# Autodesk Inventor assembly: 3d_LM-Welding_Tooling - Lathe carriage
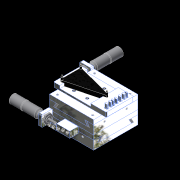
[picture p0: Inventor's stored thumbnail of the model, 180x180]
Saved by Autodesk Inventor 2018.3 (Build 223284000, 284)
## iProperties
Created: 2026-02-27
Part Number: 3d_LM-Welding_Tooling - Lathe carriage
Document SubType Name: Assembly
Designer: aca6
Author: aca6
## Documents named in this file (19)
- C:\Users\aca6\git\LM\items\3d_LM\items\LM-Welding_Tooling\3d_LM-Welding_Tooling\3d\3d_LM-Welding_Tooling - Lathe carriage.iam
- C:\Users\aca6\git\LM\items\3d_LM\items\LM-Welding_Tooling\3d_LM-Welding_Tooling\3d\3d_LM-Welding_Tooling - Adapter.ipt
- C:\Users\aca6\git\LM\items\3d_LM\items\LM-Welding_Tooling\3d_LM-Welding_Tooling\3d\3d_LM-Welding_Tooling -  Guide Pin.ipt
- C:\Users\aca6\git\LM\items\3d_LM\items\LM-Welding_Tooling\3d_LM-Welding_Tooling\3d\3d_LM-Welding_Tooling - Top Adapter.ipt
- C:\Users\aca6\git\LM\items\3d_LM\items\LM-Welding_Tooling\3d_LM-Welding_Tooling\3d\3d_LM-Welding_Tooling -  Moving Block.ipt
- C:\Users\aca6\git\LM\items\3d_LM\items\LM-Welding_Tooling\3d_LM-Welding_Tooling\3d\3d_LM-Welding_Tooling - Fixed base.ipt
- C:\Users\aca6\git\LM\items\3d_LM\items\LM-Welding_Tooling\3d_LM-Welding_Tooling\3d\3d_LM-Welding_Tooling - Acetal Stick.ipt
- C:\Users\aca6\git\LM\items\3d_LM\items\LM-Welding_Tooling\3d_LM-Welding_Tooling\3d\3d_LM-Welding_Tooling - Upper fixed base.ipt
- C:\Users\aca6\git\LM\items\3d_LM\items\LM-Welding_Tooling\3d_LM-Welding_Tooling\3d\3d_LM-Welding_Tooling - Upper moving base.ipt
- C:\Users\aca6\git\LM\items\_accesories\Tornilleria\Tornillos\3d_DIN 7991\3d\A4 Black Inox\DIN 7991 - M3x14 Black INOX.ipt
- C:\Users\aca6\git\LM\items\_accesories\Tornilleria\Tornillos\3d_DIN 7991\3d\A4 Black Inox\DIN 7991 - M3x12 Black INOX.ipt
- C:\Users\aca6\git\LM\items\3d_LM\items\LM-Welding_Tooling\3d_LM-Welding_Tooling\3d\3d_LM-Welding_Tooling -  Micrometer Nut.ipt
- C:\Users\aca6\git\LM\items\3d_LM\items\LM-Welding_Tooling\3d_LM-Welding_Tooling\3d\3d_LM-Welding_Tooling -  Micrometer.ipt
- C:\Users\aca6\git\LM\items\3d_LM\items\LM-Welding_Tooling\3d_LM-Welding_Tooling\3d\3d_LM-Welding_Tooling - Fixed Block.ipt
- C:\Users\aca6\git\LM\items\_accesories\Tornilleria\Tornillos\3d_Accu Group\3d\Prisionero nylon M4x7 REF SSN-M4-7.ipt
- C:\Users\aca6\git\LM\items\_accesories\Tornilleria\Tornillos\3d_DIN 912\3d\A4 Inox\DIN 912 - M3 x 0,5 x 8 -  INOX.ipt
- C:\Users\aca6\git\LM\items\_accesories\Tornilleria\Tornillos\3d_DIN 912\3d\A4 Inox\DIN 912 - M3 x 0,5 x 30 -  INOX.ipt
- C:\Users\aca6\git\LM\items\_accesories\Tornilleria\Tornillos\3d_DIN 912\3d\A4 Inox\DIN 912 - M3 x 0,5 x 10 -  INOX.ipt
- C:\Users\aca6\git\LM\items\3d_LM\items\LM-Welding_Tooling\3d_LM-Welding_Tooling\3d\3d_LM-Welding_Tooling - Moving base.ipt
## Components (51 placed, 18 different names)
1. 3d_LM-Welding_Tooling - Adapter:1
2. 3d_LM-Welding_Tooling -  Guide Pin:1
3. 3d_LM-Welding_Tooling -  Guide Pin:2
4. 3d_LM-Welding_Tooling -  Guide Pin:3
5. 3d_LM-Welding_Tooling - Top Adapter:1
6. 3d_LM-Welding_Tooling - Fixed base:1 — Mate:83, Flush:28, Mate:84, Flush:29
7. 3d_LM-Welding_Tooling - Acetal Stick:1 — Mate:83, Flush:28, Mate:85
8. 3d_LM-Welding_Tooling - Acetal Stick:2
9. 3d_LM-Welding_Tooling - Upper fixed base:1 — Mate:80, Mate:81, Mate:82
10. 3d_LM-Welding_Tooling - Acetal Stick:3
11. 3d_LM-Welding_Tooling - Acetal Stick:4
12. 3d_LM-Welding_Tooling - Upper moving base:1 — Flush:29
13. DIN 7991 - M3x14 Black INOX:1
14. DIN 7991 - M3x14 Black INOX:2
15. DIN 7991 - M3x14 Black INOX:3
16. DIN 7991 - M3x14 Black INOX:4
17. DIN 7991 - M3x12 Black INOX:1
18. DIN 7991 - M3x12 Black INOX:2
19. DIN 7991 - M3x12 Black INOX:3
20. DIN 7991 - M3x12 Black INOX:4
21. 3d_LM-Welding_Tooling -  Micrometer Nut:1
22. 3d_LM-Welding_Tooling -  Micrometer:1
23. 3d_LM-Welding_Tooling -  Micrometer Nut:2
24. 3d_LM-Welding_Tooling - Fixed Block:1
25. 3d_LM-Welding_Tooling -  Moving Block:3
26. Prisionero nylon M4x7 REF SSN-M4-7:1
27. Prisionero nylon M4x7 REF SSN-M4-7:2
28. Prisionero nylon M4x7 REF SSN-M4-7:3
29. Prisionero nylon M4x7 REF SSN-M4-7:4
30. 3d_LM-Welding_Tooling - Fixed Block:2
31. 3d_LM-Welding_Tooling -  Micrometer:2
32. 3d_LM-Welding_Tooling -  Moving Block:4
33. Prisionero nylon M4x7 REF SSN-M4-7:5
34. Prisionero nylon M4x7 REF SSN-M4-7:6
35. Prisionero nylon M4x7 REF SSN-M4-7:7
36. Prisionero nylon M4x7 REF SSN-M4-7:8
37. Prisionero nylon M4x7 REF SSN-M4-7:9
38. Prisionero nylon M4x7 REF SSN-M4-7:10
39. Prisionero nylon M4x7 REF SSN-M4-7:11
40. Prisionero nylon M4x7 REF SSN-M4-7:12
41. DIN 912 - M3 x 0,5 x 8 -  INOX:1
42. DIN 912 - M3 x 0,5 x 8 -  INOX:2
43. DIN 912 - M3 x 0,5 x 30 -  INOX:1 — Mate:86
44. DIN 912 - M3 x 0,5 x 30 -  INOX:2
45. DIN 912 - M3 x 0,5 x 30 -  INOX:3
46. DIN 912 - M3 x 0,5 x 30 -  INOX:4
47. DIN 912 - M3 x 0,5 x 10 -  INOX:1
48. DIN 912 - M3 x 0,5 x 10 -  INOX:2
49. DIN 912 - M3 x 0,5 x 10 -  INOX:3
50. DIN 912 - M3 x 0,5 x 10 -  INOX:4
51. 3d_LM-Welding_Tooling - Moving base:1 — Mate:80, Mate:81, Mate:82, Mate:84, Mate:85, Mate:86
## Relationships (114: Mate 79, Flush 27, Tangent 8)
- [Mate]: 3d_LM-Welding_Tooling - Adapter:1 ↔ 3d_LM-Welding_Tooling -  Guide Pin:1
- [Mate]: 3d_LM-Welding_Tooling - Adapter:1 ↔ 3d_LM-Welding_Tooling -  Guide Pin:2
- [Mate]: 3d_LM-Welding_Tooling - Adapter:1 ↔ 3d_LM-Welding_Tooling -  Guide Pin:3
- [Mate]: 3d_LM-Welding_Tooling - Adapter:1 ↔ 3d_LM-Welding_Tooling -  Guide Pin:2
- [Mate]: 3d_LM-Welding_Tooling - Adapter:1 ↔ 3d_LM-Welding_Tooling -  Guide Pin:1
- [Mate]: 3d_LM-Welding_Tooling - Adapter:1 ↔ 3d_LM-Welding_Tooling -  Guide Pin:2
- [Mate]: 3d_LM-Welding_Tooling - Adapter:1 ↔ 3d_LM-Welding_Tooling -  Guide Pin:1
- [Mate]: 3d_LM-Welding_Tooling - Adapter:1 ↔ 3d_LM-Welding_Tooling -  Guide Pin:3
- [Flush]: 3d_LM-Welding_Tooling - Adapter:1 ↔ 3d_LM-Welding_Tooling - Top Adapter:1
- [Mate]: 3d_LM-Welding_Tooling -  Guide Pin:2 ↔ 3d_LM-Welding_Tooling - Top Adapter:1
- [Mate]: 3d_LM-Welding_Tooling -  Guide Pin:1 ↔ 3d_LM-Welding_Tooling - Top Adapter:1
- [Mate]: 3d_LM-Welding_Tooling - Fixed base:1 ↔ 3d_LM-Welding_Tooling - Acetal Stick:2
- [Mate]: 3d_LM-Welding_Tooling - Fixed base:1 ↔ 3d_LM-Welding_Tooling - Acetal Stick:2
- [Flush]: 3d_LM-Welding_Tooling - Fixed base:1 ↔ 3d_LM-Welding_Tooling - Acetal Stick:1
- [Flush]: 3d_LM-Welding_Tooling - Fixed base:1 ↔ 3d_LM-Welding_Tooling - Acetal Stick:2
- [Mate]: 3d_LM-Welding_Tooling - Upper fixed base:1 ↔ 3d_LM-Welding_Tooling - Acetal Stick:3
- [Mate]: 3d_LM-Welding_Tooling - Upper fixed base:1 ↔ 3d_LM-Welding_Tooling - Acetal Stick:3
- [Mate]: 3d_LM-Welding_Tooling - Upper fixed base:1 ↔ 3d_LM-Welding_Tooling - Acetal Stick:4
- [Mate]: 3d_LM-Welding_Tooling - Upper fixed base:1 ↔ 3d_LM-Welding_Tooling - Acetal Stick:4
- [Flush]: 3d_LM-Welding_Tooling - Upper fixed base:1 ↔ 3d_LM-Welding_Tooling - Acetal Stick:4
- [Flush]: 3d_LM-Welding_Tooling - Upper fixed base:1 ↔ 3d_LM-Welding_Tooling - Acetal Stick:3
- [Mate]: 3d_LM-Welding_Tooling - Upper fixed base:1 ↔ 3d_LM-Welding_Tooling - Upper moving base:1
- [Mate]: 3d_LM-Welding_Tooling - Acetal Stick:4 ↔ 3d_LM-Welding_Tooling - Upper moving base:1
- [Mate]: 3d_LM-Welding_Tooling - Upper fixed base:1 ↔ DIN 7991 - M3x14 Black INOX:3
- [Mate]: 3d_LM-Welding_Tooling - Upper fixed base:1 ↔ DIN 7991 - M3x14 Black INOX:4
- [Mate]: 3d_LM-Welding_Tooling - Upper fixed base:1 ↔ DIN 7991 - M3x14 Black INOX:1
- [Mate]: 3d_LM-Welding_Tooling - Upper fixed base:1 ↔ DIN 7991 - M3x14 Black INOX:2
- [Tangent]: 3d_LM-Welding_Tooling - Upper fixed base:1 ↔ DIN 7991 - M3x14 Black INOX:4
- [Tangent]: 3d_LM-Welding_Tooling - Upper fixed base:1 ↔ DIN 7991 - M3x14 Black INOX:2
- [Tangent]: 3d_LM-Welding_Tooling - Upper fixed base:1 ↔ DIN 7991 - M3x14 Black INOX:1
- [Tangent]: 3d_LM-Welding_Tooling - Upper fixed base:1 ↔ DIN 7991 - M3x14 Black INOX:3
- [Mate]: 3d_LM-Welding_Tooling - Adapter:1 ↔ 3d_LM-Welding_Tooling - Upper moving base:1
- [Flush] (18.75 mm): 3d_LM-Welding_Tooling - Adapter:1 ↔ 3d_LM-Welding_Tooling - Upper moving base:1
- [Flush] (-9.684 mm): 3d_LM-Welding_Tooling - Adapter:1 ↔ 3d_LM-Welding_Tooling - Upper moving base:1
- [Mate]: 3d_LM-Welding_Tooling - Adapter:1 ↔ DIN 7991 - M3x12 Black INOX:4
- [Mate]: 3d_LM-Welding_Tooling - Adapter:1 ↔ DIN 7991 - M3x12 Black INOX:1
- [Mate]: 3d_LM-Welding_Tooling - Adapter:1 ↔ DIN 7991 - M3x12 Black INOX:3
- [Mate]: 3d_LM-Welding_Tooling - Adapter:1 ↔ DIN 7991 - M3x12 Black INOX:2
- [Tangent]: 3d_LM-Welding_Tooling - Adapter:1 ↔ DIN 7991 - M3x12 Black INOX:3
- [Tangent]: 3d_LM-Welding_Tooling - Adapter:1 ↔ DIN 7991 - M3x12 Black INOX:2
- [Tangent]: 3d_LM-Welding_Tooling - Adapter:1 ↔ DIN 7991 - M3x12 Black INOX:4
- [Tangent]: 3d_LM-Welding_Tooling - Adapter:1 ↔ DIN 7991 - M3x12 Black INOX:1
- [Mate]: 3d_LM-Welding_Tooling -  Micrometer:1 ↔ 3d_LM-Welding_Tooling - Fixed Block:1
- [Mate]: 3d_LM-Welding_Tooling -  Micrometer:1 ↔ 3d_LM-Welding_Tooling - Fixed Block:1
- [Mate]: 3d_LM-Welding_Tooling -  Micrometer:1 ↔ 3d_LM-Welding_Tooling -  Micrometer Nut:2
- [Mate]: 3d_LM-Welding_Tooling -  Micrometer Nut:2 ↔ 3d_LM-Welding_Tooling - Fixed Block:1
- [Mate]: 3d_LM-Welding_Tooling - Upper fixed base:1 ↔ 3d_LM-Welding_Tooling - Fixed Block:1
- [Flush]: 3d_LM-Welding_Tooling - Upper fixed base:1 ↔ 3d_LM-Welding_Tooling - Fixed Block:1
- [Mate]: 3d_LM-Welding_Tooling - Upper moving base:1 ↔ 3d_LM-Welding_Tooling -  Moving Block:3
- [Flush]: 3d_LM-Welding_Tooling - Upper fixed base:1 ↔ 3d_LM-Welding_Tooling - Upper moving base:1
- [Mate]: 3d_LM-Welding_Tooling - Upper fixed base:1 ↔ Prisionero nylon M4x7 REF SSN-M4-7:1
- [Mate]: 3d_LM-Welding_Tooling - Fixed base:1 ↔ Prisionero nylon M4x7 REF SSN-M4-7:2
- [Mate]: 3d_LM-Welding_Tooling - Upper fixed base:1 ↔ Prisionero nylon M4x7 REF SSN-M4-7:4
- [Mate]: 3d_LM-Welding_Tooling - Fixed base:1 ↔ Prisionero nylon M4x7 REF SSN-M4-7:3
- [Flush]: 3d_LM-Welding_Tooling - Fixed base:1 ↔ Prisionero nylon M4x7 REF SSN-M4-7:3
- [Flush]: 3d_LM-Welding_Tooling - Fixed base:1 ↔ Prisionero nylon M4x7 REF SSN-M4-7:2
- [Flush]: 3d_LM-Welding_Tooling - Upper fixed base:1 ↔ Prisionero nylon M4x7 REF SSN-M4-7:1
- [Flush]: 3d_LM-Welding_Tooling - Upper fixed base:1 ↔ Prisionero nylon M4x7 REF SSN-M4-7:4
- [Flush]: 3d_LM-Welding_Tooling - Upper fixed base:1 ↔ 3d_LM-Welding_Tooling - Fixed Block:1
- [Mate]: 3d_LM-Welding_Tooling - Fixed base:1 ↔ 3d_LM-Welding_Tooling - Fixed Block:2
- [Flush]: 3d_LM-Welding_Tooling - Fixed base:1 ↔ 3d_LM-Welding_Tooling - Fixed Block:2
- [Flush]: 3d_LM-Welding_Tooling - Fixed base:1 ↔ 3d_LM-Welding_Tooling - Fixed Block:2
- [Mate]: 3d_LM-Welding_Tooling - Fixed Block:2 ↔ 3d_LM-Welding_Tooling -  Micrometer:2
- [Mate]: 3d_LM-Welding_Tooling - Fixed Block:2 ↔ 3d_LM-Welding_Tooling -  Micrometer:2
- [Mate]: 3d_LM-Welding_Tooling -  Micrometer Nut:1 ↔ 3d_LM-Welding_Tooling -  Micrometer:2
- [Mate]: 3d_LM-Welding_Tooling -  Micrometer Nut:1 ↔ 3d_LM-Welding_Tooling - Fixed Block:2
- [Mate]: 3d_LM-Welding_Tooling - Upper moving base:1 ↔ Prisionero nylon M4x7 REF SSN-M4-7:5
- [Mate]: 3d_LM-Welding_Tooling - Upper moving base:1 ↔ Prisionero nylon M4x7 REF SSN-M4-7:8
- [Mate]: 3d_LM-Welding_Tooling - Upper moving base:1 ↔ Prisionero nylon M4x7 REF SSN-M4-7:7
- [Mate]: 3d_LM-Welding_Tooling - Upper moving base:1 ↔ Prisionero nylon M4x7 REF SSN-M4-7:6
- [Flush]: 3d_LM-Welding_Tooling - Upper moving base:1 ↔ Prisionero nylon M4x7 REF SSN-M4-7:6
- [Flush]: 3d_LM-Welding_Tooling - Upper moving base:1 ↔ Prisionero nylon M4x7 REF SSN-M4-7:5
- [Flush]: 3d_LM-Welding_Tooling - Upper moving base:1 ↔ Prisionero nylon M4x7 REF SSN-M4-7:7
- [Flush]: 3d_LM-Welding_Tooling - Upper moving base:1 ↔ Prisionero nylon M4x7 REF SSN-M4-7:8
- [Mate]: 3d_LM-Welding_Tooling - Fixed base:1 ↔ Prisionero nylon M4x7 REF SSN-M4-7:9
- [Flush]: 3d_LM-Welding_Tooling - Fixed base:1 ↔ Prisionero nylon M4x7 REF SSN-M4-7:9
- [Mate]: 3d_LM-Welding_Tooling - Fixed base:1 ↔ Prisionero nylon M4x7 REF SSN-M4-7:10
- [Flush]: 3d_LM-Welding_Tooling - Fixed base:1 ↔ Prisionero nylon M4x7 REF SSN-M4-7:10
- [Mate]: 3d_LM-Welding_Tooling - Upper fixed base:1 ↔ Prisionero nylon M4x7 REF SSN-M4-7:11
- [Flush]: 3d_LM-Welding_Tooling - Upper fixed base:1 ↔ Prisionero nylon M4x7 REF SSN-M4-7:11
- [Mate]: 3d_LM-Welding_Tooling - Upper fixed base:1 ↔ Prisionero nylon M4x7 REF SSN-M4-7:12
- [Flush]: 3d_LM-Welding_Tooling - Upper fixed base:1 ↔ Prisionero nylon M4x7 REF SSN-M4-7:12
- [Mate]: 3d_LM-Welding_Tooling -  Moving Block:4 ↔ DIN 912 - M3 x 0,5 x 8 -  INOX:2
- [Mate]: 3d_LM-Welding_Tooling -  Moving Block:4 ↔ DIN 912 - M3 x 0,5 x 8 -  INOX:2
- [Mate]: 3d_LM-Welding_Tooling -  Moving Block:3 ↔ DIN 912 - M3 x 0,5 x 8 -  INOX:1
- [Mate]: 3d_LM-Welding_Tooling -  Moving Block:3 ↔ DIN 912 - M3 x 0,5 x 8 -  INOX:1
- [Mate]: 3d_LM-Welding_Tooling -  Micrometer:2 ↔ 3d_LM-Welding_Tooling -  Moving Block:4
- [Mate]: 3d_LM-Welding_Tooling -  Micrometer:1 ↔ 3d_LM-Welding_Tooling -  Moving Block:3
- [Flush] (50 mm): 3d_LM-Welding_Tooling - Upper moving base:1 ↔ 3d_LM-Welding_Tooling -  Moving Block:3
- [Mate]: 3d_LM-Welding_Tooling -  Moving Block:4 ↔ DIN 912 - M3 x 0,5 x 30 -  INOX:2
- [Mate]: 3d_LM-Welding_Tooling -  Moving Block:4 ↔ DIN 912 - M3 x 0,5 x 30 -  INOX:1
- [Mate]: 3d_LM-Welding_Tooling -  Moving Block:4 ↔ DIN 912 - M3 x 0,5 x 30 -  INOX:2
- [Mate]: 3d_LM-Welding_Tooling -  Moving Block:4 ↔ DIN 912 - M3 x 0,5 x 30 -  INOX:1
- [Mate]: 3d_LM-Welding_Tooling -  Moving Block:3 ↔ DIN 912 - M3 x 0,5 x 30 -  INOX:3
- [Mate]: 3d_LM-Welding_Tooling -  Moving Block:3 ↔ DIN 912 - M3 x 0,5 x 30 -  INOX:4
- [Mate]: 3d_LM-Welding_Tooling -  Moving Block:3 ↔ DIN 912 - M3 x 0,5 x 30 -  INOX:4
- [Mate]: 3d_LM-Welding_Tooling -  Moving Block:3 ↔ DIN 912 - M3 x 0,5 x 30 -  INOX:3
- [Mate]: 3d_LM-Welding_Tooling - Fixed Block:1 ↔ DIN 912 - M3 x 0,5 x 10 -  INOX:2
- [Mate]: 3d_LM-Welding_Tooling - Fixed Block:1 ↔ DIN 912 - M3 x 0,5 x 10 -  INOX:1
- [Mate]: 3d_LM-Welding_Tooling - Fixed Block:1 ↔ DIN 912 - M3 x 0,5 x 10 -  INOX:1
- [Mate]: 3d_LM-Welding_Tooling - Fixed Block:1 ↔ DIN 912 - M3 x 0,5 x 10 -  INOX:2
- [Mate]: 3d_LM-Welding_Tooling - Fixed Block:2 ↔ DIN 912 - M3 x 0,5 x 10 -  INOX:4
- [Mate]: 3d_LM-Welding_Tooling - Fixed Block:2 ↔ DIN 912 - M3 x 0,5 x 10 -  INOX:3
- [Mate]: 3d_LM-Welding_Tooling - Fixed Block:2 ↔ DIN 912 - M3 x 0,5 x 10 -  INOX:3
- [Mate]: 3d_LM-Welding_Tooling - Fixed Block:2 ↔ DIN 912 - M3 x 0,5 x 10 -  INOX:4
- Mate:80: 3d_LM-Welding_Tooling - Upper fixed base:1 ↔ 3d_LM-Welding_Tooling - Moving base:1
- Mate:81: 3d_LM-Welding_Tooling - Upper fixed base:1 ↔ 3d_LM-Welding_Tooling - Moving base:1
- Mate:82: 3d_LM-Welding_Tooling - Upper fixed base:1 ↔ 3d_LM-Welding_Tooling - Moving base:1
- Mate:83: 3d_LM-Welding_Tooling - Fixed base:1 ↔ 3d_LM-Welding_Tooling - Acetal Stick:1
- Flush:28: 3d_LM-Welding_Tooling - Fixed base:1 ↔ 3d_LM-Welding_Tooling - Acetal Stick:1
- Mate:84: 3d_LM-Welding_Tooling - Fixed base:1 ↔ 3d_LM-Welding_Tooling - Moving base:1
- Mate:85: 3d_LM-Welding_Tooling - Acetal Stick:1 ↔ 3d_LM-Welding_Tooling - Moving base:1
- Flush:29: 3d_LM-Welding_Tooling - Fixed base:1 ↔ 3d_LM-Welding_Tooling - Upper moving base:1
- Mate:86: DIN 912 - M3 x 0,5 x 30 -  INOX:1 ↔ 3d_LM-Welding_Tooling - Moving base:1
## Named parameters: d236_d199 = 0 mm, d237_d201 = 0 mm, d238_d203 = 0 mm, d239_d204 = 0 mm, d90_d96 = 0 mm, d91_d97 = 0 mm, d92_d98 = 0 mm, d93_d99 = 0 mm
